# Autodesk Inventor assembly: TS_Magazin_gesamt_int
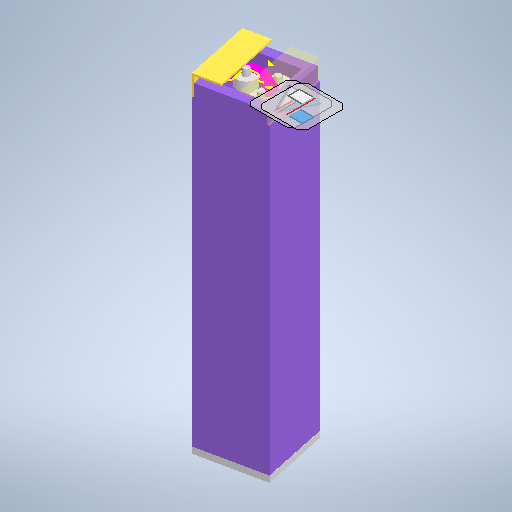
[picture p0: Inventor's stored thumbnail of the model, 512x512]
Saved by Autodesk Inventor 2025.2 (Build 292293000, 293)
## iProperties
Created: 2025-06-01
Part Number: TS_Magazin_gesamt_int
Document SubType Name: Assembly
Designer: tino
Author: tino
## Documents named in this file (13)
- C:\Users\tino\Documents_VM\Konstruieren_CAD\Useless Box\Eigene Bauteile\TS_Magazin_gesamt_int.iam
- C:\Users\tino\Documents_VM\Konstruieren_CAD\Useless Box\Eigene Bauteile\TS_Magazin_Grundplatte_int.ipt.ipt
- C:\Users\tino\Documents_VM\Konstruieren_CAD\Useless Box\Eigene Bauteile\TS_Magazin_Gehause_int.ipt
- C:\Users\tino\Documents_VM\Konstruieren_CAD\Useless Box\Eigene Bauteile\TS_Magazin_Fuehrungselement_int.ipt
- C:\Users\tino\Documents_VM\Konstruieren_CAD\Useless Box\Eigene Bauteile\TS_Magazin_Gleitbuchse_int.ipt
- C:\Users\tino\Documents_VM\Konstruieren_CAD\Useless Box\Eigene Bauteile\TS_Magazin_Begrenzung_int.ipt
- C:\Users\tino\Documents_VM\Inventor\Content Center Files\R2025\de-DE\ISO 4762(2)\ISO 4762 - M6 x 16ISO.ipt
- C:\Users\tino\Documents_VM\Inventor\Content Center Files\R2025\de-DE\ISO 4762(2)\ISO 4762 - M6 x 12ISO.ipt
- C:\Users\tino\Documents_VM\Inventor\Content Center Files\R2025\de-DE\DIN 7991(2)\DIN 7991 - M5x12.ipt
- C:\Users\tino\Documents_VM\Konstruieren_CAD\Useless Box\Eigene Bauteile\TS_Magazin_Begrenzung_int_MIR1.ipt
- C:\Users\tino\Documents_VM\Konstruieren_CAD\Useless Box\Eigene Bauteile\Feder_adaptiv.ipt
- C:\Users\tino\Documents_VM\Konstruieren_CAD\Useless Box\_Useless_Box\Finger.ipt
- TS_Magazin_Grundplatte_int.ipt
## Components (25 placed, 11 different names)
1. TS_Magazin_Grundplatte_int.ipt:1 — Passend:1, Passend:2, Passend:3, Passend:4, Passend:5, Passend:6, Passend:7, Passend:8, Passend:9, Passend:26, Passend:27, Passend:28, Passend:29, Passend:30, Passend:31, Passend:32, Passend:33, Winkel:1, Fluchtend:3, Fluchtend:11, Passend:40, Passend:41, Passend:43
2. TS_Magazin_Gehause_int:1 — Passend:7, Passend:8, Passend:9, Passend:23, Passend:24, Passend:25, Passend:34
3. TS_Magazin_Fuehrungselement_int:1 — Passend:1, Passend:6, Passend:12, Passend:37, Winkel:1, Winkel:2, Passend:44
4. TS_Magazin_Fuehrungselement_int:2 — Passend:2, Passend:5, Passend:38, Winkel:2, Winkel:3, Fluchtend:4, Fluchtend:5
5. TS_Magazin_Fuehrungselement_int:3 — Passend:3, Passend:4, Passend:36, Winkel:3
6. TS_Magazin_Gleitbuchse_int:1 — Fluchtend:1, Fluchtend:2, Passend:38, Passend:39, Winkel:4, Symmetrie:1, Fluchtend:10, Passend:40
7. TS_Magazin_Gleitbuchse_int:3 — Passend:12, Fluchtend:2, Passend:37, Winkel:4
8. TS_Magazin_Begrenzung_int:1 — Passend:23, Passend:24, Passend:25, Tangential:1, Passend:35, Tangential:2
9. ISO 4762 M6 x 12:1 — Passend:32, Passend:33
10. ISO 4762 M6 x 12:2 — Passend:30, Passend:31
11. ISO 4762 M6 x 12:3 — Passend:28, Passend:29
12. DIN 7991 M5x12:1 — Passend:35, Tangential:2
13. DIN 7991 M5x12:2 — Passend:34, Tangential:1
14. DIN 7991 M5x12:3
15. DIN 7991 M5x12:4
16. TS_Magazin_Begrenzung_int_MIR1:1
17. TS_Magazin_Gleitbuchse_int:4 — Passend:36, Fluchtend:1, Passend:42
18. Finger:1 — Passend:39, Symmetrie:1, Fluchtend:12
19. Feder_adaptiv:1 — Fluchtend:5, Fluchtend:6, Fluchtend:10, Fluchtend:11
20. Feder_adaptiv:2 — Passend:41, Passend:42
21. Feder_adaptiv:3 — Passend:43, Passend:44
22. ISO 4762 M6 x 16:1 — Passend:26, Passend:27
23. ISO 4762 M6 x 16:2
24. ISO 4762 M6 x 16:3
25. ISO 4762 M6 x 16:4
## Component patterns: (4 elements, first: ISO 4762 M6 x 16:1)
## Relationships (48: Mate 32, Flush 9, Angle 4, Tangent 2, Symmetry 1)
- Passend:1 [Mate]: TS_Magazin_Grundplatte_int.ipt:1 ↔ TS_Magazin_Fuehrungselement_int:1
- Passend:2 [Mate]: TS_Magazin_Grundplatte_int.ipt:1 ↔ TS_Magazin_Fuehrungselement_int:2
- Passend:3 [Mate]: TS_Magazin_Grundplatte_int.ipt:1 ↔ TS_Magazin_Fuehrungselement_int:3
- Passend:4 [Mate]: TS_Magazin_Grundplatte_int.ipt:1 ↔ TS_Magazin_Fuehrungselement_int:3
- Passend:5 [Mate]: TS_Magazin_Grundplatte_int.ipt:1 ↔ TS_Magazin_Fuehrungselement_int:2
- Passend:6 [Mate]: TS_Magazin_Grundplatte_int.ipt:1 ↔ TS_Magazin_Fuehrungselement_int:1
- Passend:7 [Mate]: TS_Magazin_Grundplatte_int.ipt:1 ↔ TS_Magazin_Gehause_int:1
- Passend:8 [Mate]: TS_Magazin_Grundplatte_int.ipt:1 ↔ TS_Magazin_Gehause_int:1
- Passend:9 [Mate]: TS_Magazin_Grundplatte_int.ipt:1 ↔ TS_Magazin_Gehause_int:1
- Passend:12 [Mate]: TS_Magazin_Fuehrungselement_int:1 ↔ TS_Magazin_Gleitbuchse_int:3
- Passend:23 [Mate]: TS_Magazin_Gehause_int:1 ↔ TS_Magazin_Begrenzung_int:1
- Passend:24 [Mate]: TS_Magazin_Gehause_int:1 ↔ TS_Magazin_Begrenzung_int:1
- Passend:25 [Mate]: TS_Magazin_Gehause_int:1 ↔ TS_Magazin_Begrenzung_int:1
- Passend:26 [Mate]: TS_Magazin_Grundplatte_int.ipt:1 ↔ ISO 4762 M6 x 16:1
- Passend:27 [Mate]: TS_Magazin_Grundplatte_int.ipt:1 ↔ ISO 4762 M6 x 16:1
- Passend:28 [Mate]: TS_Magazin_Grundplatte_int.ipt:1 ↔ ISO 4762 M6 x 12:3
- Passend:29 [Mate]: TS_Magazin_Grundplatte_int.ipt:1 ↔ ISO 4762 M6 x 12:3
- Passend:30 [Mate]: TS_Magazin_Grundplatte_int.ipt:1 ↔ ISO 4762 M6 x 12:2
- Passend:31 [Mate]: TS_Magazin_Grundplatte_int.ipt:1 ↔ ISO 4762 M6 x 12:2
- Passend:32 [Mate]: TS_Magazin_Grundplatte_int.ipt:1 ↔ ISO 4762 M6 x 12:1
- Passend:33 [Mate]: TS_Magazin_Grundplatte_int.ipt:1 ↔ ISO 4762 M6 x 12:1
- Passend:34 [Mate]: TS_Magazin_Gehause_int:1 ↔ DIN 7991 M5x12:2
- Tangential:1: TS_Magazin_Begrenzung_int:1 ↔ DIN 7991 M5x12:2
- Passend:35 [Mate]: TS_Magazin_Begrenzung_int:1 ↔ DIN 7991 M5x12:1
- Tangential:2: TS_Magazin_Begrenzung_int:1 ↔ DIN 7991 M5x12:1
- Passend:36 [Mate]: TS_Magazin_Fuehrungselement_int:3 ↔ TS_Magazin_Gleitbuchse_int:4
- Fluchtend:1 [Flush]: TS_Magazin_Gleitbuchse_int:1 ↔ TS_Magazin_Gleitbuchse_int:4
- Fluchtend:2 [Flush]: TS_Magazin_Gleitbuchse_int:1 ↔ TS_Magazin_Gleitbuchse_int:3
- Passend:37 [Mate]: TS_Magazin_Fuehrungselement_int:1 ↔ TS_Magazin_Gleitbuchse_int:3
- Passend:38 [Mate]: TS_Magazin_Fuehrungselement_int:2 ↔ TS_Magazin_Gleitbuchse_int:1
- Passend:39 [Mate]: TS_Magazin_Gleitbuchse_int:1 ↔ Finger:1
- Winkel:1 [Angle] (180 deg): TS_Magazin_Grundplatte_int.ipt:1 ↔ TS_Magazin_Fuehrungselement_int:1
- Winkel:2 [Angle] (0 deg): TS_Magazin_Fuehrungselement_int:1 ↔ TS_Magazin_Fuehrungselement_int:2
- Winkel:3 [Angle] (0 deg): TS_Magazin_Fuehrungselement_int:2 ↔ TS_Magazin_Fuehrungselement_int:3
- Winkel:4 [Angle] (0 deg): TS_Magazin_Gleitbuchse_int:1 ↔ TS_Magazin_Gleitbuchse_int:3
- Symmetrie:1: TS_Magazin_Gleitbuchse_int:1 ↔ Finger:1
- Fluchtend:3 [Flush]: TS_Magazin_Grundplatte_int.ipt:1
- Fluchtend:4 [Flush]: TS_Magazin_Fuehrungselement_int:2
- Fluchtend:5 [Flush]: TS_Magazin_Fuehrungselement_int:2 ↔ Feder_adaptiv:1
- Fluchtend:6 [Flush]: Feder_adaptiv:1
- Fluchtend:10 [Flush] (-12.5 mm): TS_Magazin_Gleitbuchse_int:1 ↔ Feder_adaptiv:1
- Fluchtend:11 [Flush] (-10 mm): TS_Magazin_Grundplatte_int.ipt:1 ↔ Feder_adaptiv:1
- Passend:40 [Mate] (495 mm): TS_Magazin_Grundplatte_int.ipt:1 ↔ TS_Magazin_Gleitbuchse_int:1
- Passend:41 [Mate]: TS_Magazin_Grundplatte_int.ipt:1 ↔ Feder_adaptiv:2
- Passend:42 [Mate]: TS_Magazin_Gleitbuchse_int:4 ↔ Feder_adaptiv:2
- Passend:43 [Mate]: TS_Magazin_Grundplatte_int.ipt:1 ↔ Feder_adaptiv:3
- Passend:44 [Mate]: TS_Magazin_Fuehrungselement_int:1 ↔ Feder_adaptiv:3
- Fluchtend:12 [Flush]: Finger:1
## Named parameters: springh = 507.49999 mm
